# Autodesk Inventor assembly: VersaPlanetary-1-Stage-with-BAG-Motor
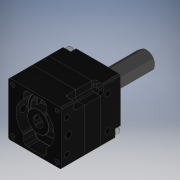
[picture p0: Inventor's stored thumbnail of the model, 180x180]
Saved by Autodesk Inventor 2016 (Build 200138000, 138)
## iProperties
Created: 2016-01-25
Part Number: VersaPlanetary-1-Stage-with-BAG-Motor
Document SubType Name: Assembly
Designer: CAD
Title: VersaPlanetary 1-Stage with BAG Motor.STEP
Description: STEP AP214
Creation Date: 2015-01-07
Sending System: SolidWorks 2014
Preprocessor: SwSTEP 2.0
Author: CAD
## Documents named in this file (10)
- C:\Users\PrashantBIA\Desktop\Robotics\Robot Assembly\Shooter\Imported Components\VersaPlanetary-1-Stage-with-BAG-Motor\VersaPlanetary-1-Stage-with-BAG-Motor.iam
- C:\Users\PrashantBIA\Desktop\Robotics\Robot Assembly\Shooter\Imported Components\VersaPlanetary-1-Stage-with-BAG-Motor\217-2742-001 Rev4.ipt
- C:\Users\PrashantBIA\Desktop\Robotics\Robot Assembly\Shooter\Imported Components\VersaPlanetary-1-Stage-with-BAG-Motor\217-2625-002 Rev1.ipt
- C:\Users\PrashantBIA\Desktop\Robotics\Robot Assembly\Shooter\Imported Components\VersaPlanetary-1-Stage-with-BAG-Motor\217-2625-018 Rev1_98541A410.ipt
- C:\Users\PrashantBIA\Desktop\Robotics\Robot Assembly\Shooter\Imported Components\VersaPlanetary-1-Stage-with-BAG-Motor\217-2625-017 Rev1_9714K61.ipt
- C:\Users\PrashantBIA\Desktop\Robotics\Robot Assembly\Shooter\Imported Components\VersaPlanetary-1-Stage-with-BAG-Motor\Ouput Shafts^VersaPlanetary_500 Hex.iam
- C:\Users\PrashantBIA\Desktop\Robotics\Robot Assembly\Shooter\Imported Components\VersaPlanetary-1-Stage-with-BAG-Motor\Input Housing^VersaPlanetary.iam
- C:\Users\PrashantBIA\Desktop\Robotics\Robot Assembly\Shooter\Imported Components\VersaPlanetary-1-Stage-with-BAG-Motor\217-2816 Rev1.iam
- C:\Users\PrashantBIA\Desktop\Robotics\Robot Assembly\Shooter\Imported Components\VersaPlanetary-1-Stage-with-BAG-Motor\217-2817 Rev1.iam
- C:\Users\PrashantBIA\Desktop\Robotics\Robot Assembly\Shooter\Imported Components\VersaPlanetary-1-Stage-with-BAG-Motor\SSA_SSA0832-1250ZC.ipt
## Components (11 placed, 11 different names)
1. 217-2742-001 Rev4_1
2. 217-2742-001 Rev4_2 — Mate:1
3. 217-2625-002 Rev1_3
4. 217-2625-018 Rev1_98541A410_4
5. 217-2625-017 Rev1_9714K61_5
6. Ouput Shafts^VersaPlanetary_500 Hex_6 [sub-assembly] — Mate:1
7. Input Housing^VersaPlanetary_8 [sub-assembly]
8. 217-2816 Rev1_9 [sub-assembly]
9. 217-2817 Rev1_10 [sub-assembly]
10. SSA_SSA0832-1250ZC_11
11. SSA_SSA0832-1250ZC_12
## Relationships (1: Mate 1)
- Mate:1: 217-2742-001 Rev4_2 ↔ Ouput Shafts^VersaPlanetary_500 Hex_6
